# Autodesk Inventor assembly: ASY PNS-002 right module
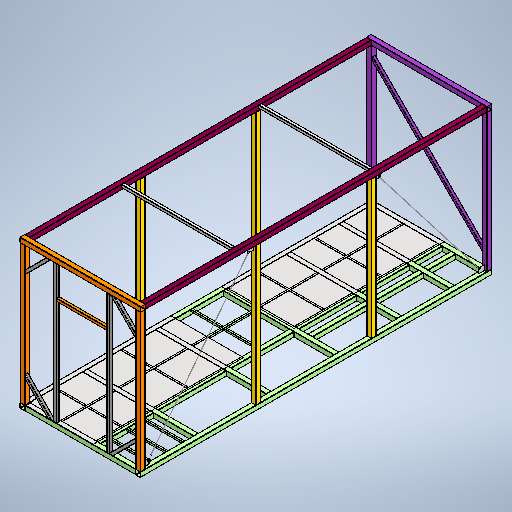
[picture p0: Inventor's stored thumbnail of the model, 512x512]
Saved by Autodesk Inventor 2025.1 (Build 291241020, 241B)
## iProperties
Created: 2025-03-25
Part Number: ASY PNS-002 right module
Document SubType Name: Assembly
Designer: user
Author: user
## Documents named in this file (10)
- C:\Users\user\YandexDisk-badmisterfox\home pc\Inventor\PNS-Panaevsk\ASY PNS-002 right module.iam
- C:\Users\user\YandexDisk-badmisterfox\home pc\Inventor\PNS-Panaevsk\ASY PNS-0210 frame right floor.iam
- C:\Users\user\YandexDisk-badmisterfox\home pc\Inventor\PNS-Panaevsk\ASY PNS-0250 frame featheredge.iam
- C:\Users\user\YandexDisk-badmisterfox\home pc\Inventor\PNS-Panaevsk\ASY PNS-0250 frame featheredge 0270.iam
- C:\Users\user\YandexDisk-badmisterfox\home pc\Inventor\PNS-Panaevsk\PNS-0261 Upper beam.ipt
- C:\Users\user\YandexDisk-badmisterfox\home pc\Inventor\PNS-Panaevsk\PNS-0262 middle pillar.ipt
- C:\Users\user\YandexDisk-badmisterfox\home pc\Inventor\PNS-Panaevsk\PNS-0262 cross beam.ipt
- C:\Users\user\YandexDisk-badmisterfox\home pc\Inventor\PNS-Panaevsk\PNS-0111 floor sheet 1.ipt
- C:\Users\user\YandexDisk-badmisterfox\home pc\Inventor\PNS-Panaevsk\PNS-071 stretch ring.ipt
- C:\Users\user\YandexDisk-badmisterfox\home pc\Inventor\PNS-Panaevsk\PNS-0310 strench.ipt
## Components (18 placed, 9 different names)
1. ASY PNS-0210 frame right floor:1 [sub-assembly] — Rigid:3, Rigid:22
2. ASY PNS-0250 frame featheredge:1 [sub-assembly] — Rigid:4, Rigid:5, Rigid:6, Rigid:7, Rigid:20
3. ASY PNS-0250 frame featheredge 0270:1 [sub-assembly] — Rigid:3, Rigid:8, Rigid:9, Rigid:21
4. PNS-0261 Upper beam:1 — Rigid:4, Mate:5, Flush:3, Mate:6, Flush:4
5. PNS-0261 Upper beam:2 — Rigid:5
6. PNS-0262 middle pillar:1 — Rigid:6, Rigid:19
7. PNS-0262 middle pillar:2 — Rigid:7
8. PNS-0262 middle pillar:3 — Rigid:8, Rigid:18
9. PNS-0262 middle pillar:4 — Rigid:9
10. PNS-0262 cross beam:1 — Mate:6, Flush:4
11. PNS-0262 cross beam:2 — Mate:5, Flush:3
12. PNS-0111 floor sheet 1:1 — Rigid:22
13. PNS-071 stretch ring:1 — Rigid:19
14. PNS-071 stretch ring:2 — Rigid:20
15. PNS-0310 strench:1
16. PNS-071 stretch ring:3 — Rigid:18
17. PNS-071 stretch ring:4 — Rigid:21
18. PNS-0310 strench:2
## Relationships (21: WeldJoint 13, Mate 4, Flush 4)
- [WeldJoint]: ASY PNS-0210 frame right floor:1 ↔ ASY PNS-0250 frame featheredge:1
- Rigid:3 [WeldJoint]: ASY PNS-0210 frame right floor:1 ↔ ASY PNS-0250 frame featheredge 0270:1
- Rigid:4 [WeldJoint] (-100 mm): ASY PNS-0250 frame featheredge:1 ↔ PNS-0261 Upper beam:1
- Rigid:5 [WeldJoint] (-100 mm): ASY PNS-0250 frame featheredge:1 ↔ PNS-0261 Upper beam:2
- Rigid:6 [WeldJoint] (2200 mm): ASY PNS-0250 frame featheredge:1 ↔ PNS-0262 middle pillar:1
- Rigid:7 [WeldJoint] (2200 mm): ASY PNS-0250 frame featheredge:1 ↔ PNS-0262 middle pillar:2
- Rigid:8 [WeldJoint] (2200 mm): ASY PNS-0250 frame featheredge 0270:1 ↔ PNS-0262 middle pillar:3
- Rigid:9 [WeldJoint] (2200 mm): ASY PNS-0250 frame featheredge 0270:1 ↔ PNS-0262 middle pillar:4
- [Mate]: PNS-071 stretch ring:1 ↔ PNS-0310 strench:1
- [Flush]: PNS-071 stretch ring:1 ↔ PNS-0310 strench:1
- [Mate]: PNS-071 stretch ring:3 ↔ PNS-0310 strench:2
- [Flush]: PNS-071 stretch ring:3 ↔ PNS-0310 strench:2
- Rigid:18 [WeldJoint]: PNS-0262 middle pillar:3 ↔ PNS-071 stretch ring:3
- Rigid:19 [WeldJoint]: PNS-0262 middle pillar:1 ↔ PNS-071 stretch ring:1
- Rigid:20 [WeldJoint]: ASY PNS-0250 frame featheredge:1 ↔ PNS-071 stretch ring:2
- Rigid:21 [WeldJoint]: ASY PNS-0250 frame featheredge 0270:1 ↔ PNS-071 stretch ring:4
- Rigid:22 [WeldJoint]: ASY PNS-0210 frame right floor:1 ↔ PNS-0111 floor sheet 1:1
- Mate:5: PNS-0261 Upper beam:1 ↔ PNS-0262 cross beam:2
- Flush:3: PNS-0261 Upper beam:1 ↔ PNS-0262 cross beam:2
- Mate:6: PNS-0261 Upper beam:1 ↔ PNS-0262 cross beam:1
- Flush:4: PNS-0261 Upper beam:1 ↔ PNS-0262 cross beam:1
## Named parameters: d18_d19 = 0 mm, d22_d20 = 0 mm
